# Autodesk Inventor assembly: New_Odom_Assembly
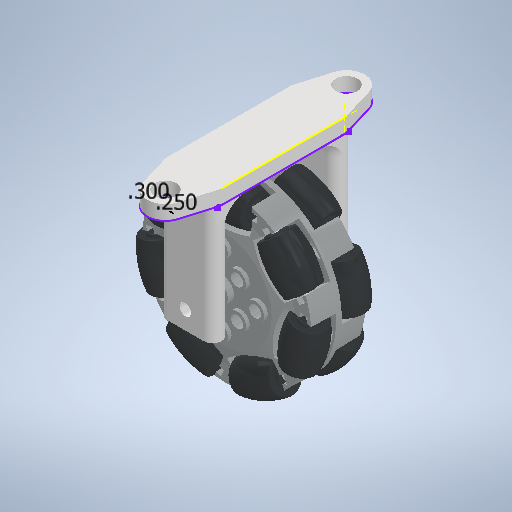
[picture p0: Inventor's stored thumbnail of the model, 512x512]
Saved by Autodesk Inventor 2025.1 (Build 291241020, 241B)
## iProperties
Created: 2024-11-18
Part Number: New_Odom_Assembly
Document SubType Name: Assembly
Designer: AtuStem
Author: AtuStem
## Documents named in this file (3)
- C:\Users\AtuStem\Documents\GitHub\ATUM-V5RC-High-Stakes-CAD\Odometers_Collin\New_Odom_Assembly.iam
- C:\Users\AtuStem\Documents\GitHub\ATUM-V5RC-High-Stakes-CAD\Odometers_Collin\IQ_OMNI.iam
- C:\Users\AtuStem\Documents\GitHub\ATUM-V5RC-High-Stakes-CAD\Odometers_Collin\Latest_Odom.ipt
## Components (2 placed, 2 different names)
1. Latest_Odom:1 — Mate:1
2. IQ_OMNI:1 [sub-assembly] — Mate:1
## Relationships (1: Mate 1)
- Mate:1: Latest_Odom:1 ↔ IQ_OMNI:1
